# Autodesk Inventor assembly: Nanopower_plus_BP4
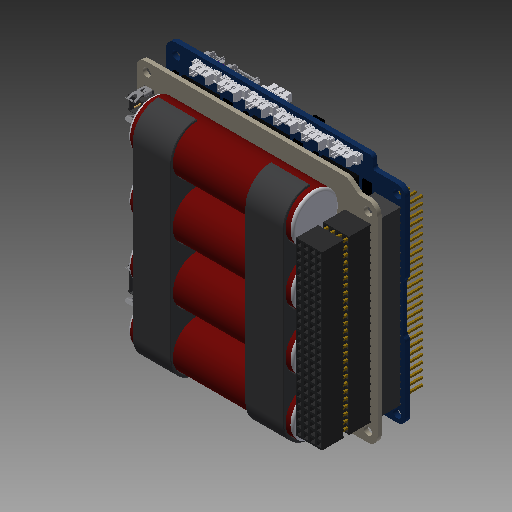
[picture p0: Inventor's stored thumbnail of the model, 512x512]
Saved by Autodesk Inventor 2017 (Build 210142000, 142)
## iProperties
Created: 2016-03-16
Part Number: Nanopower_plus_BP4
Document SubType Name: Assembly
Designer: Cosmonauta
Author: Cosmonauta
## Documents named in this file (3)
- C:\Users\Cosmonauta\ownCloud\Aurora\Proyectos\SUCHAI_2-3\Subsistemas\MEC\CAD_Cubesat3U\Nanopower_plus_BP4\Nanopower_plus_BP4.iam
- C:\Users\Cosmonauta\ownCloud\Aurora\Proyectos\SUCHAI_2-3\Subsistemas\MEC\CAD_Cubesat3U\Nanopower_P31U\CAD\NanoPower P31u-9.iam
- C:\Users\Cosmonauta\ownCloud\Aurora\Proyectos\SUCHAI_2-3\Subsistemas\MEC\CAD_Cubesat3U\Nanopower_BP4\CAD\bp4-2.0.iam
## Components (2 placed, 2 different names)
1. NanoPower P31u-9:1 [sub-assembly] — Mate:1, Mate:2, Mate:3
2. bp4-2.0:1 [sub-assembly] — Mate:1, Mate:2, Mate:3
## Relationships (3: Mate 3)
- Mate:1 (10 mm): NanoPower P31u-9:1 ↔ bp4-2.0:1
- Mate:2: NanoPower P31u-9:1 ↔ bp4-2.0:1
- Mate:3: NanoPower P31u-9:1 ↔ bp4-2.0:1
